# Autodesk Inventor assembly: Assembly19
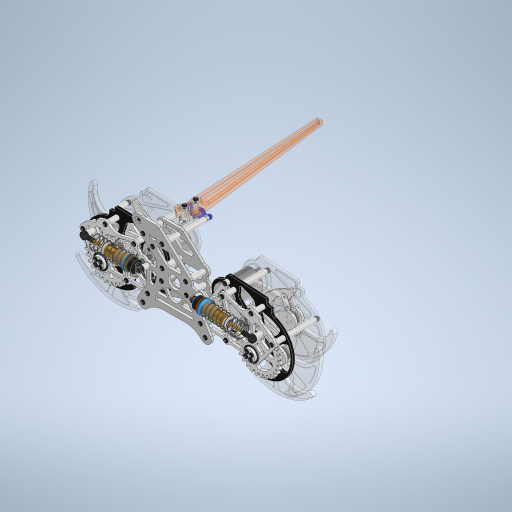
[picture p0: Inventor's stored thumbnail of the model, 512x512]
Saved by Autodesk Inventor 2023 (Build 270158000, 158)
## iProperties
Created: 2022-06-23
Part Number: Assembly19
Document SubType Name: Assembly
Designer: muzho
Mass: 885.534 g
Surface Area: 2969.65 cm^2
Volume: 326.998 cm^3
Density: 2.70807 g/cm^3
Author: muzho
## Documents named in this file (7)
- C:\Users\muzho\Documents\srdc\srdc_2\脚\足全体_反対.iam
- C:\Users\muzho\Documents\srdc\srdc_2\脚\足ユニット.iam
- C:\Users\muzho\Documents\srdc\srdc_2\脚\MIR\足ユニット_MIR.iam
- C:\Users\muzho\Documents\srdc\srdc_2\脚\MIR\中間ユニット_MIR.iam
- C:\Users\muzho\Documents\srdc\srdc_2\スペーサ\l10.ipt
- C:\Users\muzho\Documents\srdc\srdc_2\タミヤダンパー1.iam
- C:\Users\muzho\Documents\srdc\srdc_2\スペーサ\l7.ipt
## Components (9 placed, 6 different names)
1. 足ユニット:1 [sub-assembly] — メイト:2, 挿入:1
2. 足ユニット_MIR:1 [sub-assembly] — メイト:1, 挿入:2
3. 中間ユニット_MIR:1 [sub-assembly] — メイト:1, メイト:2, 挿入:3, 挿入:4
4. l10:1 — 挿入:1, 挿入:6
5. l10:2 — 挿入:2, 挿入:8
6. タミヤダンパー1:1 [sub-assembly] — 挿入:5, 挿入:6
7. タミヤダンパー1:2 [sub-assembly] — 挿入:7, 挿入:8
8. l7:1 — 挿入:3, 挿入:5
9. l7:2 — 挿入:4, 挿入:7
## Relationships (10: Insert 8, Mate 2)
- メイト:1 [Mate]: 足ユニット_MIR:1 ↔ 中間ユニット_MIR:1
- メイト:2 [Mate]: 足ユニット:1 ↔ 中間ユニット_MIR:1
- 挿入:1 [Insert]: 足ユニット:1 ↔ l10:1
- 挿入:2 [Insert]: 足ユニット_MIR:1 ↔ l10:2
- 挿入:3 [Insert]: 中間ユニット_MIR:1 ↔ l7:1
- 挿入:4 [Insert]: 中間ユニット_MIR:1 ↔ l7:2
- 挿入:5 [Insert]: タミヤダンパー1:1 ↔ l7:1
- 挿入:6 [Insert]: l10:1 ↔ タミヤダンパー1:1
- 挿入:7 [Insert]: タミヤダンパー1:2 ↔ l7:2
- 挿入:8 [Insert]: l10:2 ↔ タミヤダンパー1:2
